# Autodesk Inventor assembly: Assembly
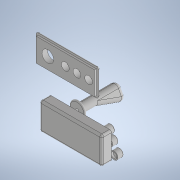
[picture p0: Inventor's stored thumbnail of the model, 180x180]
Saved by Autodesk Inventor 2021 (Build 250183000, 183)
## iProperties
Created: 2021-03-26
Part Number: Assembly
Document SubType Name: Assembly
Designer: eng1-139
Author: eng1-139
## Documents named in this file (6)
- C:\Users\eng1-139\Desktop\Assembly.iam
- C:\Users\eng1-139\Downloads\Device Base.ipt
- C:\Users\eng1-139\Downloads\Device Joystick.ipt
- C:\Users\eng1-139\Desktop\Mon-46 Controller\Device Direction Button.ipt
- C:\Users\eng1-139\Desktop\Mon-46 Controller\Device Rotation Button.ipt
- C:\Users\eng1-139\Desktop\Mon-46 Controller\Device Top Cover.ipt
## Components (6 placed, 5 different names)
1. Device Base:1 — Ball:1
2. Device Joystick:1 — Ball:1
3. Device Direction Button:1
4. Device Direction Button:2
5. Device Rotation Button:1
6. Device Top Cover:1
## Relationships (1: BallJoint 1)
- Ball:1: Device Base:1 ↔ Device Joystick:1
